# Autodesk Inventor assembly: Gesamtzusammensetzung
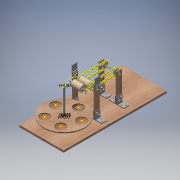
[picture p0: Inventor's stored thumbnail of the model, 180x180]
Saved by Autodesk Inventor 2018 (Build 220112000, 112)
## iProperties
Created: 2018-03-14
Part Number: Gesamtzusammensetzung
Material: Generisch
Document SubType Name: Assembly
Designer: Julian
Author: Julian
## Documents named in this file (4)
- C:\Users\Julian\Desktop\Schule\5AHME\Diplomarbeit\Git\fuettr_prototype\Mechanical\Inventorskizzen\Gesamtzusammensetzung.iam
- C:\Users\Julian\Desktop\Schule\5AHME\Diplomarbeit\Git\fuettr_prototype\Mechanical\Inventorskizzen\Grundplatte.ipt
- C:\Users\Julian\Desktop\Schule\5AHME\Diplomarbeit\Git\fuettr_prototype\Mechanical\Inventorskizzen\Plattenzusammensetzung.iam
- C:\Users\Julian\Desktop\Schule\5AHME\Diplomarbeit\Git\fuettr_prototype\Mechanical\Inventorskizzen\Förderband.iam
## Components (3 placed, 3 different names)
1. Grundplatte:2 — Drehbar:1, Drehbar:2
2. Plattenzusammensetzung:1 [sub-assembly] — Drehbar:1
3. Förderband:1 [sub-assembly] — Drehbar:2
## Relationships (2: RevoluteJoint 2)
- Drehbar:1 [RevoluteJoint]: Grundplatte:2 ↔ Plattenzusammensetzung:1
- Drehbar:2 [RevoluteJoint]: Grundplatte:2 ↔ Förderband:1
